# Autodesk Inventor assembly: 500mm_X95_with_base_and_clamp
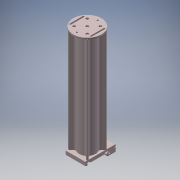
[picture p0: Inventor's stored thumbnail of the model, 180x180]
Saved by Autodesk Inventor 2016 (Build 200138000, 138)
## iProperties
Created: 2018-09-27
Part Number: 500mm_X95_with_base_and_clamp
Document SubType Name: Assembly
Designer: voigt
Author: voigt
## Documents named in this file (4)
- D:\Microscope_Design\CAD_Files\mesoSPIM_design\mesoSPIM\sample_stages\500mm_X95_with_base_and_clamp.iam
- D:\Microscope_Design\CAD_Files\mesoSPIM_design\library\Qioptiq\X95_accessoires\X95_baseplate.ipt
- D:\Microscope_Design\CAD_Files\mesoSPIM_design\library\Qioptiq\X95_rails\X95_500mm.ipt
- D:\Microscope_Design\CAD_Files\mesoSPIM_design\library\Qioptiq\X95_carriers\X95_clamping_carrier.ipt
## Components (3 placed, 3 different names)
1. X95_baseplate:1 — Mate:1, Mate:2, Mate:3
2. X95_500mm:1 — Mate:1, Mate:2, Mate:3, Mate:4, Mate:5, Mate:6
3. X95_clamping_carrier:1 — Mate:4, Mate:5, Mate:6
## Relationships (6: Mate 6)
- Mate:1: X95_baseplate:1 ↔ X95_500mm:1
- Mate:2: X95_baseplate:1 ↔ X95_500mm:1
- Mate:3: X95_baseplate:1 ↔ X95_500mm:1
- Mate:4: X95_500mm:1 ↔ X95_clamping_carrier:1
- Mate:5: X95_500mm:1 ↔ X95_clamping_carrier:1
- Mate:6: X95_500mm:1 ↔ X95_clamping_carrier:1
